# Autodesk Inventor assembly: Battery_holder_WZY-148-1_with_cable
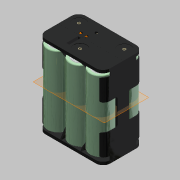
[picture p0: Inventor's stored thumbnail of the model, 180x180]
Saved by Autodesk Inventor 2019.3 (Build 233278000, 278)
## iProperties
Created: 2019-02-20
Part Number: Battery_holder_WZY-148-1_with_cable
Document SubType Name: Assembly
Designer: Varga Daniel
Author: Varga Daniel
## Documents named in this file (3)
- C:\!_Dani\!_cloud\OneDrive\!_munka\Revolution\RevvyDemoKit\Structural parts\Demo parts\Battery\Inventor Imported\Battery_holder_WZY-148-1_with_cable.iam
- C:\!_Dani\!_cloud\OneDrive\!_munka\Revolution\RevvyDemoKit\Structural parts\Demo parts\Battery\Inventor Imported\Battery_holder_WZY-148-1.ipt
- C:\!_Dani\!_cloud\OneDrive\!_munka\Revolution\RevvyDemoKit\Structural parts\Demo parts\Battery\Inventor Imported\Battery.ipt
## Components (7 placed, 2 different names)
1. Battery_holder_WZY-148-1:1 — Mate:2, Mate:4, Mate:6, Mate:8, Mate:10, Mate:12, Tangent:1, Tangent:2, Tangent:3, Tangent:4, Tangent:5, Tangent:6, Tangent:7, Tangent:8, Tangent:9, Tangent:10, Tangent:11, Tangent:12
2. Battery:1 — Mate:2, Tangent:11, Tangent:12
3. Battery:2 — Mate:4, Tangent:1, Tangent:2
4. Battery:3 — Mate:8, Tangent:9, Tangent:10
5. Battery:4 — Mate:10, Tangent:7, Tangent:8
6. Battery:5 — Mate:12, Tangent:5, Tangent:6
7. Battery:6 — Mate:6, Tangent:3, Tangent:4
## Relationships (18: Tangent 12, Mate 6)
- Mate:2: Battery_holder_WZY-148-1:1 ↔ Battery:1
- Mate:4: Battery_holder_WZY-148-1:1 ↔ Battery:2
- Mate:6: Battery_holder_WZY-148-1:1 ↔ Battery:6
- Mate:8: Battery_holder_WZY-148-1:1 ↔ Battery:3
- Mate:10: Battery_holder_WZY-148-1:1 ↔ Battery:4
- Mate:12: Battery_holder_WZY-148-1:1 ↔ Battery:5
- Tangent:1: Battery_holder_WZY-148-1:1 ↔ Battery:2
- Tangent:2: Battery_holder_WZY-148-1:1 ↔ Battery:2
- Tangent:3: Battery_holder_WZY-148-1:1 ↔ Battery:6
- Tangent:4: Battery_holder_WZY-148-1:1 ↔ Battery:6
- Tangent:5: Battery_holder_WZY-148-1:1 ↔ Battery:5
- Tangent:6: Battery_holder_WZY-148-1:1 ↔ Battery:5
- Tangent:7: Battery_holder_WZY-148-1:1 ↔ Battery:4
- Tangent:8: Battery_holder_WZY-148-1:1 ↔ Battery:4
- Tangent:9: Battery_holder_WZY-148-1:1 ↔ Battery:3
- Tangent:10: Battery_holder_WZY-148-1:1 ↔ Battery:3
- Tangent:11: Battery_holder_WZY-148-1:1 ↔ Battery:1
- Tangent:12: Battery_holder_WZY-148-1:1 ↔ Battery:1
